# Autodesk Inventor assembly: S3x1
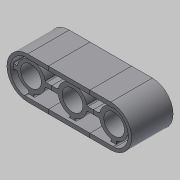
[picture p0: Inventor's stored thumbnail of the model, 180x180]
Saved by Autodesk Inventor 2020 (Build 240168000, 168)
## iProperties
Created: 2019-04-27
Part Number: S3x1
Document SubType Name: Assembly
Designer: Varga Daniel
Author: Varga Daniel
## Documents named in this file (4)
- C:\!_Dani\!_cloud\OneDrive\!_munka\Revolution\StructuralParts\Beams\Straight Beams\S1+x1\S3x1.iam
- C:\!_Dani\!_cloud\OneDrive\!_munka\Revolution\StructuralParts\Beams\beam_single_end_part.ipt
- C:\!_Dani\!_cloud\OneDrive\!_munka\Revolution\StructuralParts\Beams\beam_single_inner_part.ipt
- C:\!_Dani\!_cloud\OneDrive\!_munka\Revolution\StructuralParts\Beams\Straight Beams\S1+x1.iam
## Components (3 placed, 2 different names)
1. beam_single_end_part:1 — Flush:1, Flush:2, Flush:3, Flush:4, End_part_mate, Flush:5, Mate:2, Flush:6, Flush:7
2. beam_single_end_part:2 — Flush:4, End_part_mate, Flush:5
3. beam_single_inner_part:1 — Mate:2, Flush:6, Flush:7
## Component patterns: (1 elements, first: beam_single_inner_part:1)
## Relationships (9: Flush 7, Mate 2)
- Flush:1: beam_single_end_part:1
- Flush:2: beam_single_end_part:1
- Flush:3: beam_single_end_part:1
- Flush:4: beam_single_end_part:1 ↔ beam_single_end_part:2
- End_part_mate [Mate] (10 mm): beam_single_end_part:1 ↔ beam_single_end_part:2
- Flush:5: beam_single_end_part:1 ↔ beam_single_end_part:2
- Mate:2: beam_single_end_part:1 ↔ beam_single_inner_part:1
- Flush:6: beam_single_end_part:1 ↔ beam_single_inner_part:1
- Flush:7: beam_single_end_part:1 ↔ beam_single_inner_part:1
